# Autodesk Inventor assembly: Montagem2
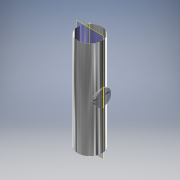
[picture p0: Inventor's stored thumbnail of the model, 180x180]
Saved by Autodesk Inventor 2016 (Build 200138000, 138)
## iProperties
Created: 2017-04-03
Part Number: Montagem2
Document SubType Name: Assembly
Designer: Marcelo
Author: Marcelo
## Documents named in this file (3)
- D:\Users\Marcelo\Documents\GitHub\telescopiocaseiro\Hardware\PT-001\Montagem2.iam
- D:\Users\Marcelo\Documents\GitHub\telescopiocaseiro\Hardware\PT-001\Tubo.ipt
- D:\Users\Marcelo\Documents\GitHub\telescopiocaseiro\Hardware\PT-001\DiscoSuporteInterno.ipt
## Components (3 placed, 2 different names)
1. Tubo:1 — Mate:1, Mate:4, Mate:5, Mate:7
2. DiscoSuporteInterno:1 — Mate:1, Mate:4, Mate:6
3. DiscoSuporteInterno:2 — Mate:5, Mate:6, Mate:7
## Relationships (5: Mate 5)
- Mate:1: Tubo:1 ↔ DiscoSuporteInterno:1
- Mate:4 (-400 mm): Tubo:1 ↔ DiscoSuporteInterno:1
- Mate:5: Tubo:1 ↔ DiscoSuporteInterno:2
- Mate:6: DiscoSuporteInterno:1 ↔ DiscoSuporteInterno:2
- Mate:7: Tubo:1 ↔ DiscoSuporteInterno:2
